# Autodesk Inventor assembly: Train_001
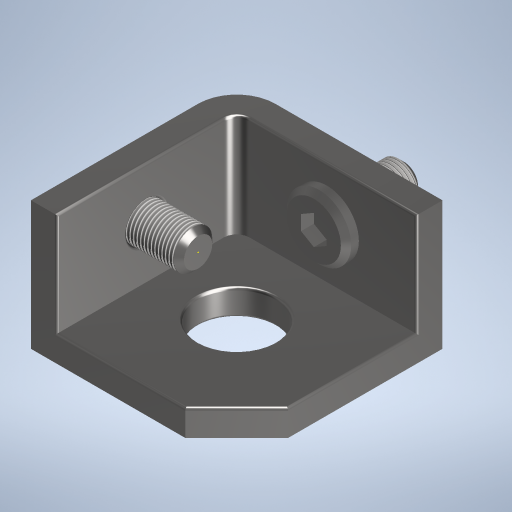
[picture p0: Inventor's stored thumbnail of the model, 512x512]
Saved by Autodesk Inventor 2024.3 (Build 283343000, 343)
## iProperties
Created: 2026-06-11
Part Number: Train_001
Document SubType Name: Assembly
Designer: scott
Author: scott
## Documents named in this file (3)
- C:\Users\scott\OneDrive\Documents\GitHub\2026-2027-DesignTraining\Scott\Train_001.iam
- C:\Users\scott\OneDrive\Documents\GitHub\2026-2027-DesignTraining\Scott\Train_002_PracticeBracket.ipt
- C:\Users\scott\OneDrive\Documents\GitHub\2026-2027-DesignTraining\Scott\Train_003_PracticeBolt.ipt
## Components (3 placed, 2 different names)
1. Train_002_PracticeBracket:1 — Mate:1, Mate:2, Mate:3, Mate:4
2. Train_003_PracticeBolt:1 — Mate:1, Mate:2
3. Train_003_PracticeBolt:2 — Mate:3, Mate:4
## Relationships (4: Mate 4)
- Mate:1: Train_002_PracticeBracket:1 ↔ Train_003_PracticeBolt:1
- Mate:2: Train_002_PracticeBracket:1 ↔ Train_003_PracticeBolt:1
- Mate:3: Train_002_PracticeBracket:1 ↔ Train_003_PracticeBolt:2
- Mate:4: Train_002_PracticeBracket:1 ↔ Train_003_PracticeBolt:2
